# Autodesk Inventor assembly: Finger Assembly Left
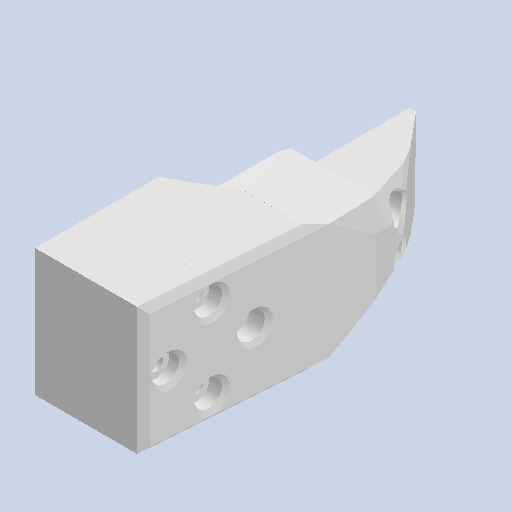
[picture p0: Inventor's stored thumbnail of the model, 512x512]
Saved by Autodesk Inventor 2022 (Build 260153000, 153)
## iProperties
Created: 2021-09-24
Part Number: Finger Assembly Left
Document SubType Name: Assembly
Designer: kylem
Author: kylem
## Documents named in this file (3)
- C:\Users\kylem\OneDrive\Documents\GitHub\IMML_Contactile_Gripper_Hardware\Finger Assembly Left.iam
- C:\Users\kylem\OneDrive\Documents\GitHub\IMML_Contactile_Gripper_Hardware\Contactile Sensor.ipt
- C:\Users\kylem\OneDrive\Documents\GitHub\IMML_Contactile_Gripper_Hardware\Finger_left.ipt
## Components (2 placed, 2 different names)
1. Contactile Sensor:1 — Mate:1, Mate:2, Flush:1
2. Finger_left:1 — Mate:1, Mate:2, Flush:1
## Relationships (3: Mate 2, Flush 1)
- Mate:1: Contactile Sensor:1 ↔ Finger_left:1
- Mate:2: Contactile Sensor:1 ↔ Finger_left:1
- Flush:1: Contactile Sensor:1 ↔ Finger_left:1
